# Autodesk Inventor assembly: 21015-22-1-0- Overall weldment assembly
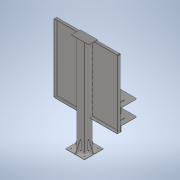
[picture p0: Inventor's stored thumbnail of the model, 180x180]
Saved by Autodesk Inventor 2022 (Build 260153000, 153)
## iProperties
Created: 2021-06-17
Part Number: 21015-22-1-0- Overall weldment assembly
Document SubType Name: Weldment
Designer: Skynet
Weld Material: Welded Aluminum-6061
Author: Skynet
## Documents named in this file (7)
- C:\Users\Skynet\Downloads\weldment assembly\New folder\21015-22-1-0- Overall weldment assembly.iam
- C:\Users\Skynet\Downloads\weldment assembly\New folder\21015-22-1-1- Floor Plate.ipt
- C:\Users\Skynet\Downloads\weldment assembly\New folder\21015-22-1-3- 6X6 Stanchion.ipt
- C:\Users\Skynet\Downloads\weldment assembly\New folder\21015-22-1-4- Back Panel.ipt
- C:\Users\Skynet\Downloads\weldment assembly\New folder\21015-22-1-5- Manifold mounting plate.ipt
- C:\Users\Skynet\Downloads\weldment assembly\New folder\21015-22-1-6- Work Shelves.ipt
- C:\Users\Skynet\Downloads\weldment assembly\New folder\21015-22-1-2- Floor Plate Gussets.ipt
## Components (10 placed, 6 different names)
1. 21015-22-1-1- Floor Plate:1 — Mate:1, Mate:2, Mate:3, Mate:9, Mate:12, Mate:14, Mate:16
2. 21015-22-1-3- 6X6 Stanchion:1 — Mate:1, Mate:2, Mate:3, Mate:4, Mate:5, Flush:1, Mate:6, Mate:10, Flush:8, Flush:9, Mate:11, Mate:13, Flush:10, Mate:15, Flush:11
3. 21015-22-1-4- Back Panel:1 — Mate:4, Mate:5, Flush:1, Flush:2, Flush:3, Mate:7, Flush:4, Flush:5, Mate:8, Flush:7
4. 21015-22-1-5- Manifold mounting plate:1 — Flush:2, Mate:6, Flush:3
5. 21015-22-1-6- Work Shelves:1 — Mate:7, Flush:4, Flush:5, Flush:6
6. 21015-22-1-6- Work Shelves:2 — Flush:6, Mate:8, Flush:7
7. 21015-22-1-2- Floor Plate Gussets:1 — Mate:9, Mate:10, Flush:8
8. 21015-22-1-2- Floor Plate Gussets:2 — Mate:13, Flush:10, Mate:14
9. 21015-22-1-2- Floor Plate Gussets:3 — Flush:9, Mate:11, Mate:12
10. 21015-22-1-2- Floor Plate Gussets:4 — Mate:15, Mate:16, Flush:11
## Relationships (27: Mate 16, Flush 11)
- Mate:1 (101.6 mm): 21015-22-1-1- Floor Plate:1 ↔ 21015-22-1-3- 6X6 Stanchion:1
- Mate:2: 21015-22-1-1- Floor Plate:1 ↔ 21015-22-1-3- 6X6 Stanchion:1
- Mate:3 (101.6 mm): 21015-22-1-1- Floor Plate:1 ↔ 21015-22-1-3- 6X6 Stanchion:1
- Mate:4: 21015-22-1-3- 6X6 Stanchion:1 ↔ 21015-22-1-4- Back Panel:1
- Mate:5 (1.27 mm): 21015-22-1-3- 6X6 Stanchion:1 ↔ 21015-22-1-4- Back Panel:1
- Flush:1: 21015-22-1-3- 6X6 Stanchion:1 ↔ 21015-22-1-4- Back Panel:1
- Flush:2: 21015-22-1-4- Back Panel:1 ↔ 21015-22-1-5- Manifold mounting plate:1
- Mate:6: 21015-22-1-3- 6X6 Stanchion:1 ↔ 21015-22-1-5- Manifold mounting plate:1
- Flush:3 (444.5 mm): 21015-22-1-4- Back Panel:1 ↔ 21015-22-1-5- Manifold mounting plate:1
- Mate:7: 21015-22-1-4- Back Panel:1 ↔ 21015-22-1-6- Work Shelves:1
- Flush:4 (6.35 mm): 21015-22-1-4- Back Panel:1 ↔ 21015-22-1-6- Work Shelves:1
- Flush:5: 21015-22-1-4- Back Panel:1 ↔ 21015-22-1-6- Work Shelves:1
- Flush:6 (-298.45 mm): 21015-22-1-6- Work Shelves:1 ↔ 21015-22-1-6- Work Shelves:2
- Mate:8: 21015-22-1-4- Back Panel:1 ↔ 21015-22-1-6- Work Shelves:2
- Flush:7: 21015-22-1-4- Back Panel:1 ↔ 21015-22-1-6- Work Shelves:2
- Mate:9: 21015-22-1-1- Floor Plate:1 ↔ 21015-22-1-2- Floor Plate Gussets:1
- Mate:10: 21015-22-1-3- 6X6 Stanchion:1 ↔ 21015-22-1-2- Floor Plate Gussets:1
- Flush:8 (71.4375 mm): 21015-22-1-3- 6X6 Stanchion:1 ↔ 21015-22-1-2- Floor Plate Gussets:1
- Flush:9 (71.4375 mm): 21015-22-1-3- 6X6 Stanchion:1 ↔ 21015-22-1-2- Floor Plate Gussets:3
- Mate:11: 21015-22-1-3- 6X6 Stanchion:1 ↔ 21015-22-1-2- Floor Plate Gussets:3
- Mate:12: 21015-22-1-1- Floor Plate:1 ↔ 21015-22-1-2- Floor Plate Gussets:3
- Mate:13: 21015-22-1-3- 6X6 Stanchion:1 ↔ 21015-22-1-2- Floor Plate Gussets:2
- Flush:10 (71.4375 mm): 21015-22-1-3- 6X6 Stanchion:1 ↔ 21015-22-1-2- Floor Plate Gussets:2
- Mate:14: 21015-22-1-1- Floor Plate:1 ↔ 21015-22-1-2- Floor Plate Gussets:2
- Mate:15: 21015-22-1-3- 6X6 Stanchion:1 ↔ 21015-22-1-2- Floor Plate Gussets:4
- Mate:16: 21015-22-1-1- Floor Plate:1 ↔ 21015-22-1-2- Floor Plate Gussets:4
- Flush:11 (71.4375 mm): 21015-22-1-3- 6X6 Stanchion:1 ↔ 21015-22-1-2- Floor Plate Gussets:4
